# Autodesk Inventor assembly: Framing_For_First_Floor_Back_Bathroom_Window
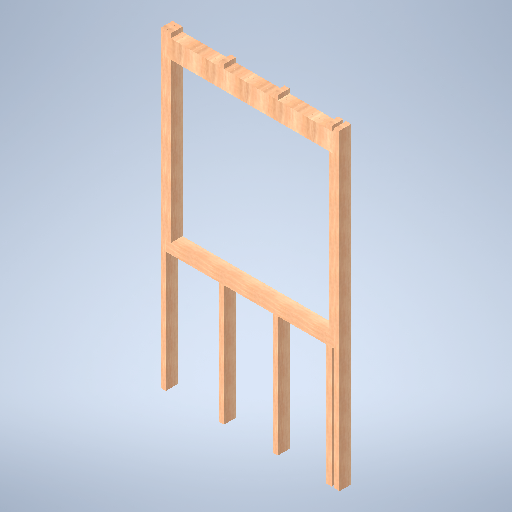
[picture p0: Inventor's stored thumbnail of the model, 512x512]
Saved by Autodesk Inventor 2025 (Build 290162010, 162A)
## iProperties
Created: 2024-09-15
Part Number: Framing_For_First_Floor_Back_Bathroom_Window
Document SubType Name: Assembly
Designer: Tom
Author: Tom
## Documents named in this file (7)
- C:\Users\Tom\Documents\Inventor\Mobility\Additional_Building\Framing_For_Bathroom_Window.iam
- C:\Users\Tom\Documents\Inventor\Mobility\Additional_Building\Stud_With_Height_93_Inches.ipt
- C:\Users\Tom\Documents\Inventor\Mobility\Additional_Building\Stud_With_Height_35.9375_Inches.ipt
- C:\Users\Tom\Documents\Inventor\Mobility\Additional_Building\Sill_Plate_With_Length_50.25_Inches.ipt
- C:\Users\Tom\Documents\Inventor\Mobility\Additional_Building\Stud_With_Height_47.25_Inches.ipt
- C:\Users\Tom\Documents\Inventor\Mobility\Additional_Building\Stud_With_Height_1.3125_Inches.ipt
- C:\Users\Tom\Documents\Inventor\Mobility\Additional_Building\Header_With_Dimensions_3.5_x_5.5_x_50.25_Inches.iam
## Components (14 placed, 6 different names)
1. Stud_With_Height_93_Inches:62 — Mate:64, Flush:74, Flush:75, Mate:65, Mate:68, Flush:81, Flush:83, Flush:84, Flush:89, Mate:75, Flush:91, Flush:93, Mate:78
2. Sill_Plate_With_Length_50.25_Inches:1 — Mate:64, Flush:74, Flush:75, Mate:66, Flush:76, Mate:73, Flush:82, Flush:84, Flush:85, Flush:88
3. Sill_Plate_With_Length_50.25_Inches:2 — Mate:65, Mate:66, Flush:76, Mate:67, Flush:77, Mate:71, Flush:79, Flush:80, Flush:85, Flush:86
4. Stud_With_Height_47.25_Inches:1 — Mate:67, Flush:77, Mate:68, Flush:86, Mate:74
5. Stud_With_Height_47.25_Inches:2 — Mate:71, Flush:79, Flush:80, Mate:72
6. Stud_With_Height_93_Inches:63 — Mate:72, Flush:81, Flush:88
7. Header_With_Dimensions_3.5_x_5.5_x_50.25_Inches:1 [sub-assembly] — Mate:74, Mate:75, Flush:91, Mate:76, Flush:92, Mate:77
8. Stud_With_Height_1.3125_Inches:4 — Mate:77, Flush:93, Mate:78
9. Stud_With_Height_35.9375_Inches:1 — Mate:73, Flush:82, Flush:89, Flush:90
10. Stud_With_Height_1.3125_Inches:1 — Flush:83, Flush:90, Flush:92
11. Stud_With_Height_35.9375_Inches:2
12. Stud_With_Height_1.3125_Inches:2
13. Stud_With_Height_35.9375_Inches:3
14. Stud_With_Height_1.3125_Inches:3 — Mate:76
## Component patterns: (3 elements, first: Stud_With_Height_35.9375_Inches:1 + Stud_With_Height_1.3125_Inches:1)
## Relationships (31: Flush 18, Mate 13)
- Mate:64: Stud_With_Height_93_Inches:62 ↔ Sill_Plate_With_Length_50.25_Inches:1
- Flush:74: Stud_With_Height_93_Inches:62 ↔ Sill_Plate_With_Length_50.25_Inches:1
- Flush:75 (912.8125 mm): Stud_With_Height_93_Inches:62 ↔ Sill_Plate_With_Length_50.25_Inches:1
- Mate:65: Stud_With_Height_93_Inches:62 ↔ Sill_Plate_With_Length_50.25_Inches:2
- Mate:66: Sill_Plate_With_Length_50.25_Inches:1 ↔ Sill_Plate_With_Length_50.25_Inches:2
- Flush:76: Sill_Plate_With_Length_50.25_Inches:1 ↔ Sill_Plate_With_Length_50.25_Inches:2
- Mate:67: Sill_Plate_With_Length_50.25_Inches:2 ↔ Stud_With_Height_47.25_Inches:1
- Flush:77: Sill_Plate_With_Length_50.25_Inches:2 ↔ Stud_With_Height_47.25_Inches:1
- Mate:68: Stud_With_Height_93_Inches:62 ↔ Stud_With_Height_47.25_Inches:1
- Mate:71: Sill_Plate_With_Length_50.25_Inches:2 ↔ Stud_With_Height_47.25_Inches:2
- Flush:79: Sill_Plate_With_Length_50.25_Inches:2 ↔ Stud_With_Height_47.25_Inches:2
- Flush:80: Sill_Plate_With_Length_50.25_Inches:2 ↔ Stud_With_Height_47.25_Inches:2
- Mate:72: Stud_With_Height_47.25_Inches:2 ↔ Stud_With_Height_93_Inches:63
- Flush:81: Stud_With_Height_93_Inches:62 ↔ Stud_With_Height_93_Inches:63
- Mate:73: Sill_Plate_With_Length_50.25_Inches:1 ↔ Stud_With_Height_35.9375_Inches:1
- Flush:82: Sill_Plate_With_Length_50.25_Inches:1 ↔ Stud_With_Height_35.9375_Inches:1
- Flush:83: Stud_With_Height_93_Inches:62 ↔ Stud_With_Height_1.3125_Inches:1
- Flush:84: Stud_With_Height_93_Inches:62 ↔ Sill_Plate_With_Length_50.25_Inches:1
- Flush:85: Sill_Plate_With_Length_50.25_Inches:1 ↔ Sill_Plate_With_Length_50.25_Inches:2
- Flush:86: Sill_Plate_With_Length_50.25_Inches:2 ↔ Stud_With_Height_47.25_Inches:1
- Flush:88: Sill_Plate_With_Length_50.25_Inches:1 ↔ Stud_With_Height_93_Inches:63
- Flush:89 (441.325 mm): Stud_With_Height_93_Inches:62 ↔ Stud_With_Height_35.9375_Inches:1
- Flush:90: Stud_With_Height_35.9375_Inches:1 ↔ Stud_With_Height_1.3125_Inches:1
- Mate:74: Stud_With_Height_47.25_Inches:1 ↔ Header_With_Dimensions_3.5_x_5.5_x_50.25_Inches:1
- Mate:75: Stud_With_Height_93_Inches:62 ↔ Header_With_Dimensions_3.5_x_5.5_x_50.25_Inches:1
- Flush:91: Stud_With_Height_93_Inches:62 ↔ Header_With_Dimensions_3.5_x_5.5_x_50.25_Inches:1
- Mate:76: Header_With_Dimensions_3.5_x_5.5_x_50.25_Inches:1 ↔ Stud_With_Height_1.3125_Inches:3
- Flush:92: Header_With_Dimensions_3.5_x_5.5_x_50.25_Inches:1 ↔ Stud_With_Height_1.3125_Inches:1
- Mate:77: Header_With_Dimensions_3.5_x_5.5_x_50.25_Inches:1 ↔ Stud_With_Height_1.3125_Inches:4
- Flush:93: Stud_With_Height_93_Inches:62 ↔ Stud_With_Height_1.3125_Inches:4
- Mate:78: Stud_With_Height_93_Inches:62 ↔ Stud_With_Height_1.3125_Inches:4
